# Autodesk Inventor assembly: Soporte
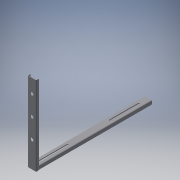
[picture p0: Inventor's stored thumbnail of the model, 180x180]
Saved by Autodesk Inventor 2016 (Build 200138000, 138)
## iProperties
Created: 2015-11-10
Part Number: Soporte
Document SubType Name: Weldment
Designer: serge
Weld Material: Steel, Carbon
Author: serge
## Documents named in this file (3)
- D:\Programas\xampp\htdocs\localUnal\storage\macros\cuarto\Modelado\Soporte Unidades\Soporte.iam
- D:\Programas\xampp\htdocs\localUnal\storage\macros\cuarto\Modelado\Soporte Unidades\Soporte Horizontal.ipt
- D:\Programas\xampp\htdocs\localUnal\storage\macros\cuarto\Modelado\Soporte Unidades\Soporte vertical.ipt
## Components (2 placed, 2 different names)
1. Soporte Horizontal:1 — Mate:1, Flush:1, Mate:2
2. Soporte vertical:1 — Mate:1, Flush:1, Mate:2
## Relationships (3: Mate 2, Flush 1)
- Mate:1: Soporte Horizontal:1 ↔ Soporte vertical:1
- Flush:1: Soporte Horizontal:1 ↔ Soporte vertical:1
- Mate:2: Soporte Horizontal:1 ↔ Soporte vertical:1
